# Autodesk Inventor assembly: LeapMotionAssembly
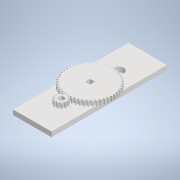
[picture p0: Inventor's stored thumbnail of the model, 180x180]
Saved by Autodesk Inventor 2022 (Build 260153000, 153)
## iProperties
Created: 2021-09-18
Part Number: LeapMotionAssembly
Document SubType Name: Assembly
Designer: marcu
Author: marcu
## Documents named in this file (4)
- C:\Users\marcu\OneDrive\Documents\Pinncale\3DPrinting\LeapMotionAssembly\LeapMotionAssembly.iam
- C:\Users\marcu\OneDrive\Documents\Pinncale\3DPrinting\LeapMotionAssembly\Board.ipt
- C:\Users\marcu\OneDrive\Documents\Pinncale\3DPrinting\LeapMotionAssembly\Gear1.ipt
- C:\Users\marcu\OneDrive\Documents\Pinncale\3DPrinting\LeapMotionAssembly\Gear2.ipt
## Components (3 placed, 3 different names)
1. Board:1 — Mate:1, Mate:2, Insert:1
2. Gear1:1 — Mate:1, Mate:2
3. Gear2:1 — Insert:1
## Relationships (3: Mate 2, Insert 1)
- Mate:1: Board:1 ↔ Gear1:1
- Mate:2: Board:1 ↔ Gear1:1
- Insert:1: Board:1 ↔ Gear2:1
